# Autodesk Inventor assembly: pablogilLCDCase
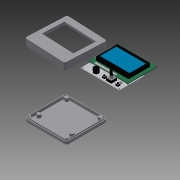
[picture p0: Inventor's stored thumbnail of the model, 180x180]
Saved by Autodesk Inventor 2015 SP1 (Build 190203100, 203)
## iProperties
Created: 2015-04-16
Part Number: pablogilLCDCase
Document SubType Name: Assembly
Designer: Jack
Author: Jack
## Documents named in this file (4)
- C:\Users\Jack\ownCloud\Projects\CrossBot\InventorModel\Enclosure\LCDCase\pablogilLCDCase.iam
- C:\Users\Jack\ownCloud\Projects\CrossBot\InventorModel\Electronics\LCD\GLCDKnockoff.ipt
- C:\Users\Jack\ownCloud\Projects\CrossBot\InventorModel\Enclosure\LCDCase\LCDDerivativeBottom1.ipt
- C:\Users\Jack\ownCloud\Projects\CrossBot\InventorModel\Enclosure\LCDCase\LCDDerivativeTop1.ipt
## Components (3 placed, 3 different names)
1. GLCDKnockoff:1 — Mate:1
2. LCDDerivativeBottom1:1 — Mate:2
3. LCDDerivativeTop1:1 — Mate:1, Mate:2
## Relationships (2: Mate 2)
- Mate:1: GLCDKnockoff:1 ↔ LCDDerivativeTop1:1
- Mate:2: LCDDerivativeBottom1:1 ↔ LCDDerivativeTop1:1
